# Autodesk Inventor assembly: twoPmtDetector
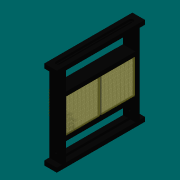
[picture p0: Inventor's stored thumbnail of the model, 180x180]
Saved by Autodesk Inventor 2016 SP1 (Build 200210100, 210)
## iProperties
Created: 2016-04-02
Part Number: twoPmtDetector
Document SubType Name: Assembly
Designer: sawai
Author: sawai
## Documents named in this file (5)
- C:\Users\sawai\OneDrive\projects\modularRICH\detector\twoPmtDetector.iam
- C:\Users\sawai\OneDrive\projects\modularRICH\detector\detectorArray.iam
- C:\Users\sawai\OneDrive\projects\modularRICH\detector\detectorSuppourt.ipt
- C:\Users\sawai\OneDrive\projects\modularRICH\detector\verticalSupourt.ipt
- C:\Users\sawai\OneDrive\projects\modularRICH\detector\horizontalSupourt.ipt
## Components (7 placed, 4 different names)
1. detectorArray:1 [sub-assembly] — Flush:2, Mate:1, Mate:2, Flush:3
2. detectorSuppourt:1 — Flush:1, Flush:2, Mate:1, Flush:4, Symmetry:2
3. detectorSuppourt:2 — Flush:1, Mate:2, Flush:3, Flush:4, Mate:3, Flush:5, Flush:6, Mate:4, Symmetry:2
4. verticalSupourt:1 — Mate:3, Flush:5, Flush:7, Flush:8, Flush:9, Mate:11, Symmetry:1
5. verticalSupourt:2 — Flush:6, Mate:4, Flush:7, Mate:10, Symmetry:1
6. horizontalSupourt:1 — Flush:8, Mate:10, Flush:10, Symmetry:3, Symmetry:4, Symmetry:5
7. horizontalSupourt:2 — Flush:9, Mate:11, Flush:10, Symmetry:3, Symmetry:4, Symmetry:5
## Relationships (21: Flush 10, Mate 6, Symmetry 5)
- Flush:1: detectorSuppourt:1 ↔ detectorSuppourt:2
- Flush:2: detectorArray:1 ↔ detectorSuppourt:1
- Mate:1: detectorArray:1 ↔ detectorSuppourt:1
- Mate:2: detectorArray:1 ↔ detectorSuppourt:2
- Flush:3: detectorArray:1 ↔ detectorSuppourt:2
- Flush:4: detectorSuppourt:1 ↔ detectorSuppourt:2
- Mate:3: detectorSuppourt:2 ↔ verticalSupourt:1
- Flush:5: detectorSuppourt:2 ↔ verticalSupourt:1
- Flush:6: detectorSuppourt:2 ↔ verticalSupourt:2
- Mate:4: detectorSuppourt:2 ↔ verticalSupourt:2
- Flush:7: verticalSupourt:1 ↔ verticalSupourt:2
- Flush:8: verticalSupourt:1 ↔ horizontalSupourt:1
- Mate:10: verticalSupourt:2 ↔ horizontalSupourt:1
- Flush:9: verticalSupourt:1 ↔ horizontalSupourt:2
- Mate:11: verticalSupourt:1 ↔ horizontalSupourt:2
- Symmetry:1: verticalSupourt:1 ↔ verticalSupourt:2
- Symmetry:2: detectorSuppourt:1 ↔ detectorSuppourt:2
- Flush:10: horizontalSupourt:1 ↔ horizontalSupourt:2
- Symmetry:3: horizontalSupourt:1 ↔ horizontalSupourt:2
- Symmetry:4: horizontalSupourt:1 ↔ horizontalSupourt:2
- Symmetry:5: horizontalSupourt:1 ↔ horizontalSupourt:2
